# Autodesk Inventor assembly: MeasurementChamber V4 - Assembly - Bade
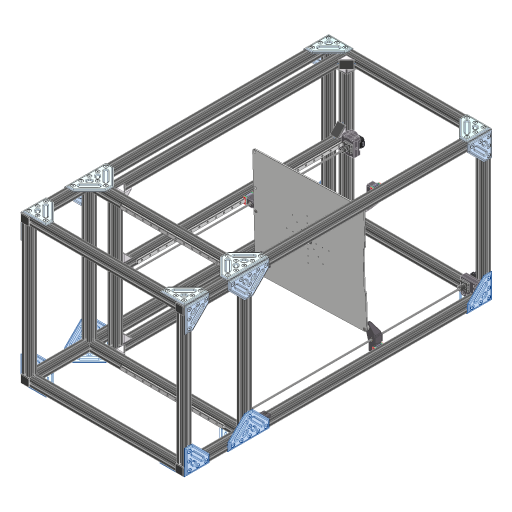
[picture p0: Inventor's stored thumbnail of the model, 512x512]
Saved by Autodesk Inventor 2023 (Build 270158000, 158)
## iProperties
Created: 2024-02-07
Part Number: MeasurementChamber V4 - Assembly - Bade
Document SubType Name: Assembly
Designer: Nils Bade
Author: Nils Bade
## Documents named in this file (12)
- C:\Users\Nils Bade\Documents\Projektarbeit_Bade\GIT\Masterarbeit-Inventor\Abbildungen-Dokumentation\Bed-Misalignment_Measurements.iam
- C:\Users\Nils Bade\Documents\Projektarbeit_Bade\GIT\Masterarbeit-Inventor\ITEM\ITEM Frame Assembly - Bade v1.iam
- ITEM Frame Assembly - Bade v1.iam
- C:\Users\Nils Bade\Documents\Projektarbeit_Bade\GIT\Masterarbeit-Inventor\RatRig_Bade\Z-Axis Transmission Assembly Back.iam
- C:\Users\Nils Bade\Documents\Projektarbeit_Bade\GIT\Masterarbeit-Inventor\RatRig_Bade\Z-Axis Transmission Assembly Front.iam
- C:\Users\Nils Bade\Documents\Projektarbeit_Bade\GIT\Masterarbeit-Inventor\RatRig_modified\Lead Screw - TR8x8-2p 1057mm Simple.ipt
- C:\Users\Nils Bade\Documents\Projektarbeit_Bade\GIT\Masterarbeit-Inventor\RatRig_modified\Leadscrew Constraint Front for 4040 - Assembly.iam
- C:\Users\Nils Bade\Documents\Projektarbeit_Bade\GIT\Masterarbeit-Inventor\RatRig_modified\Leadscrew Constraint Rear for 4040 - Assembly.iam
- C:\Users\Nils Bade\Documents\Projektarbeit_Bade\GIT\Masterarbeit-Inventor\RatRig_Bade\Bed Arm Back for 4040 - Assembly.iam
- C:\Users\Nils Bade\Documents\Projektarbeit_Bade\GIT\Masterarbeit-Inventor\RatRig_Bade\Bed Arm Left for 4040 - Assembly.iam
- C:\Users\Nils Bade\Documents\Projektarbeit_Bade\GIT\Masterarbeit-Inventor\RatRig_Bade\Bed Arm Right for 4040 - Assembly.iam
- C:\Users\Nils Bade\Documents\Projektarbeit_Bade\GIT\Masterarbeit-Inventor\RatRig_Bade\RatRig-Bade-BedAssembly.iam
## Components (14 placed, 10 different names)
1. ITEM Frame Assembly - Bade v1:1 [sub-assembly] — Passend:1, Passend:2, Passend:3, Passend:4, Passend:5, Passend:6, Passend:7, Passend:8, Passend:9, Passend:10, Passend:11, Passend:12, Passend:16, Passend:17, Passend:18, Passend:19, Passend:20, Passend:21, Passend:22, Fluchtend:3, Fluchtend:4, Passend:23, Passend:24, Passend:26
2. RatRig-Bade-BedAssembly:1 [sub-assembly] — Passend:30, Passend:31, Passend:32
3. Z-Axis Transmission Assembly Back:1 [sub-assembly] — Passend:1, Passend:2, Passend:3, Passend:15
4. Z-Axis Transmission Assembly Front:1 [sub-assembly] — Passend:4, Passend:5, Passend:6, Passend:14
5. Z-Axis Transmission Assembly Front:2 [sub-assembly] — Passend:7, Passend:8, Passend:9, Passend:13
6. LeadScrew - TR8x8-2p 1057mm Simple:1 — Passend:10, Passend:15, Passend:25
7. LeadScrew - TR8x8-2p 1057mm Simple:2 — Passend:11, Passend:14
8. LeadScrew - TR8x8-2p 1057mm Simple:3 — Passend:12, Passend:13
9. Leadscrew Constraint Front for 4040 - Assembly:1 [sub-assembly] — Passend:16, Passend:19, Fluchtend:1, Passend:22
10. Leadscrew Constraint Front for 4040 - Assembly:2 [sub-assembly] — Passend:17, Passend:18, Fluchtend:1, Fluchtend:2
11. Leadscrew Constraint Rear for 4040 - Assembly:1 [sub-assembly] — Passend:20, Passend:21, Fluchtend:2
12. Bed Arm Back for 4040 - Assembly:1 [sub-assembly] — Fluchtend:3, Passend:25, Passend:31
13. Bed Arm Left for 4040 - Assembly:1 [sub-assembly] — Passend:23, Passend:26, Passend:30
14. Bed Arm Right for 4040 - Assembly:1 [sub-assembly] — Fluchtend:4, Passend:24, Passend:32
## Relationships (33: Mate 29, Flush 4)
- Passend:1 [Mate]: ITEM Frame Assembly - Bade v1:1 ↔ Z-Axis Transmission Assembly Back:1
- Passend:2 [Mate]: ITEM Frame Assembly - Bade v1:1 ↔ Z-Axis Transmission Assembly Back:1
- Passend:3 [Mate]: ITEM Frame Assembly - Bade v1:1 ↔ Z-Axis Transmission Assembly Back:1
- Passend:4 [Mate]: ITEM Frame Assembly - Bade v1:1 ↔ Z-Axis Transmission Assembly Front:1
- Passend:5 [Mate]: ITEM Frame Assembly - Bade v1:1 ↔ Z-Axis Transmission Assembly Front:1
- Passend:6 [Mate]: ITEM Frame Assembly - Bade v1:1 ↔ Z-Axis Transmission Assembly Front:1
- Passend:7 [Mate]: ITEM Frame Assembly - Bade v1:1 ↔ Z-Axis Transmission Assembly Front:2
- Passend:8 [Mate]: ITEM Frame Assembly - Bade v1:1 ↔ Z-Axis Transmission Assembly Front:2
- Passend:9 [Mate]: ITEM Frame Assembly - Bade v1:1 ↔ Z-Axis Transmission Assembly Front:2
- Passend:10 [Mate]: ITEM Frame Assembly - Bade v1:1 ↔ LeadScrew - TR8x8-2p 1057mm Simple:1
- Passend:11 [Mate]: ITEM Frame Assembly - Bade v1:1 ↔ LeadScrew - TR8x8-2p 1057mm Simple:2
- Passend:12 [Mate]: ITEM Frame Assembly - Bade v1:1 ↔ LeadScrew - TR8x8-2p 1057mm Simple:3
- Passend:13 [Mate]: Z-Axis Transmission Assembly Front:2 ↔ LeadScrew - TR8x8-2p 1057mm Simple:3
- Passend:14 [Mate]: Z-Axis Transmission Assembly Front:1 ↔ LeadScrew - TR8x8-2p 1057mm Simple:2
- Passend:15 [Mate]: Z-Axis Transmission Assembly Back:1 ↔ LeadScrew - TR8x8-2p 1057mm Simple:1
- Passend:16 [Mate]: ITEM Frame Assembly - Bade v1:1 ↔ Leadscrew Constraint Front for 4040 - Assembly:1
- Passend:17 [Mate]: ITEM Frame Assembly - Bade v1:1 ↔ Leadscrew Constraint Front for 4040 - Assembly:2
- Passend:18 [Mate]: ITEM Frame Assembly - Bade v1:1 ↔ Leadscrew Constraint Front for 4040 - Assembly:2
- Passend:19 [Mate]: ITEM Frame Assembly - Bade v1:1 ↔ Leadscrew Constraint Front for 4040 - Assembly:1
- Fluchtend:1 [Flush]: Leadscrew Constraint Front for 4040 - Assembly:1 ↔ Leadscrew Constraint Front for 4040 - Assembly:2
- Passend:20 [Mate]: ITEM Frame Assembly - Bade v1:1 ↔ Leadscrew Constraint Rear for 4040 - Assembly:1
- Passend:21 [Mate]: ITEM Frame Assembly - Bade v1:1 ↔ Leadscrew Constraint Rear for 4040 - Assembly:1
- Fluchtend:2 [Flush]: Leadscrew Constraint Front for 4040 - Assembly:2 ↔ Leadscrew Constraint Rear for 4040 - Assembly:1
- Passend:22 [Mate] (5 mm): ITEM Frame Assembly - Bade v1:1 ↔ Leadscrew Constraint Front for 4040 - Assembly:1
- Fluchtend:3 [Flush]: ITEM Frame Assembly - Bade v1:1 ↔ Bed Arm Back for 4040 - Assembly:1
- Fluchtend:4 [Flush]: ITEM Frame Assembly - Bade v1:1 ↔ Bed Arm Right for 4040 - Assembly:1
- Passend:23 [Mate]: ITEM Frame Assembly - Bade v1:1 ↔ Bed Arm Left for 4040 - Assembly:1
- Passend:24 [Mate]: ITEM Frame Assembly - Bade v1:1 ↔ Bed Arm Right for 4040 - Assembly:1
- Passend:25 [Mate]: LeadScrew - TR8x8-2p 1057mm Simple:1 ↔ Bed Arm Back for 4040 - Assembly:1
- Passend:26 [Mate]: ITEM Frame Assembly - Bade v1:1 ↔ Bed Arm Left for 4040 - Assembly:1
- Passend:30 [Mate] (0.6 mm): RatRig-Bade-BedAssembly:1 ↔ Bed Arm Left for 4040 - Assembly:1
- Passend:31 [Mate] (0.6 mm): RatRig-Bade-BedAssembly:1 ↔ Bed Arm Back for 4040 - Assembly:1
- Passend:32 [Mate] (0.6 mm): RatRig-Bade-BedAssembly:1 ↔ Bed Arm Right for 4040 - Assembly:1
